# Autodesk Inventor assembly: s-assy-guide_actuator
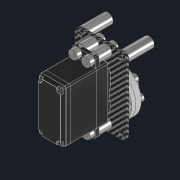
[picture p0: Inventor's stored thumbnail of the model, 180x180]
Saved by Autodesk Inventor 2022 (Build 260153000, 153)
## iProperties
Created: 2021-08-27
Part Number: s-assy-guide_actuator
Document SubType Name: Assembly
Designer: Yuta Kage
Author: Yuta Kage
## Documents named in this file (9)
- C:\Users\yuta0\Documents\GitHub\catchrobo_hardware\assy-shooter\s-assy-guide_actuator.iam
- C:\Users\yuta0\Documents\GitHub\catchrobo_hardware\assy-shooter\s_base5.ipt
- C:\Users\yuta0\Documents\GitHub\catchrobo_hardware\assy-robot\CB3-10.ipt
- C:\Users\yuta0\Documents\GitHub\catchrobo_hardware\assy-shooter\s_base6.ipt
- C:\Users\yuta0\Documents\GitHub\catchrobo_hardware\assy-shooter\SCSTR6-8.iam
- C:\Users\yuta0\Documents\GitHub\catchrobo_hardware\assy-robot\LBNR3.ipt
- C:\Users\yuta0\Documents\GitHub\catchrobo_hardware\assy-shooter\CB3-6.ipt
- C:\Users\yuta0\Documents\GitHub\catchrobo_hardware\assy-robot\ARF-420E.ipt
- C:\Users\yuta0\Documents\GitHub\catchrobo_hardware\assy-shooter\s-assy-shooter_motor.iam
## Components (31 placed, 8 different names)
1. s_base5:1 — メイト:4, メイト:5, メイト:9, メイト:13, メイト:14, メイト:15, メイト:37, メイト:38
2. s_base6:1 — メイト:6, メイト:7, メイト:9, メイト:11, メイト:12, メイト:13, メイト:16, メイト:17, メイト:39, メイト:40
3. SCSTR6-8:1 [sub-assembly] — メイト:6, メイト:7, メイト:40
4. ARF-420E:1 — メイト:33, メイト:34
5. ARF-420E:2 — メイト:32, メイト:36
6. ARF-420E:3 — メイト:31, メイト:35
7. s-assy-shooter_motor:1 [sub-assembly] — メイト:31, メイト:32, メイト:33, メイト:34, メイト:35, メイト:36, メイト:37, メイト:38
8. CB3-6:1 — メイト:4, メイト:5
9. CB3-10:5 — メイト:11, メイト:12
10. CB3-6:2
11. CB3-10:6
12. CB3-6:3
13. CB3-10:7
14. CB3-6:4
15. CB3-10:8
16. LBNR3:1 — メイト:14, メイト:15
17. CB3-10:9 — メイト:16, メイト:17
18. LBNR3:2
19. CB3-10:10
20. LBNR3:3
21. CB3-10:11
22. LBNR3:4
23. CB3-10:12
24. LBNR3:5
25. CB3-10:13
26. LBNR3:6
27. CB3-10:14
28. LBNR3:7
29. CB3-10:15
30. LBNR3:8
31. CB3-10:16
## Component patterns: (4 elements, first: CB3-6:1 + CB3-10:5), (8 elements, first: LBNR3:1 + CB3-10:9)
## Relationships (22: Mate 22)
- メイト:4 [Mate]: s_base5:1 ↔ CB3-6:1
- メイト:5 [Mate]: s_base5:1 ↔ CB3-6:1
- メイト:6 [Mate]: s_base6:1 ↔ SCSTR6-8:1
- メイト:7 [Mate]: s_base6:1 ↔ SCSTR6-8:1
- メイト:9 [Mate]: s_base5:1 ↔ s_base6:1
- メイト:11 [Mate]: s_base6:1 ↔ CB3-10:5
- メイト:12 [Mate]: s_base6:1 ↔ CB3-10:5
- メイト:13 [Mate]: s_base5:1 ↔ s_base6:1
- メイト:14 [Mate]: s_base5:1 ↔ LBNR3:1
- メイト:15 [Mate]: s_base5:1 ↔ LBNR3:1
- メイト:16 [Mate]: s_base6:1 ↔ CB3-10:9
- メイト:17 [Mate]: s_base6:1 ↔ CB3-10:9
- メイト:31 [Mate]: ARF-420E:3 ↔ s-assy-shooter_motor:1
- メイト:32 [Mate]: ARF-420E:2 ↔ s-assy-shooter_motor:1
- メイト:33 [Mate]: ARF-420E:1 ↔ s-assy-shooter_motor:1
- メイト:34 [Mate]: ARF-420E:1 ↔ s-assy-shooter_motor:1
- メイト:35 [Mate]: ARF-420E:3 ↔ s-assy-shooter_motor:1
- メイト:36 [Mate]: ARF-420E:2 ↔ s-assy-shooter_motor:1
- メイト:37 [Mate]: s_base5:1 ↔ s-assy-shooter_motor:1
- メイト:38 [Mate]: s_base5:1 ↔ s-assy-shooter_motor:1
- メイト:39 [Mate]: s_base6:1
- メイト:40 [Mate]: s_base6:1 ↔ SCSTR6-8:1
